# Autodesk Inventor assembly: Assemblyarm
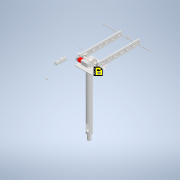
[picture p0: Inventor's stored thumbnail of the model, 180x180]
Saved by Autodesk Inventor 2022 (Build 260153000, 153)
## iProperties
Created: 2022-02-06
Part Number: Assemblyarm
Document SubType Name: Assembly
Designer: pauly
Author: pauly
## Documents named in this file (17)
- C:\Users\pauly\OneDrive\Documents\Robotics arm\Assemblyarm.iam
- C:\Users\pauly\OneDrive\Documents\Robotics arm\Shaft connecting chassis updated 1-19.ipt
- C:\Users\pauly\OneDrive\Documents\Robotics arm\base_plate.ipt
- C:\Users\pauly\OneDrive\Documents\Robotics arm\Updated Support.ipt
- C:\Users\pauly\OneDrive\Documents\Robotics arm\am-2986 FR8ZZ Hex Bearing.ipt
- C:\Users\pauly\OneDrive\Documents\Robotics arm\am-0856 500 Hex Shaft for Modulox REV3.ipt
- C:\Users\pauly\OneDrive\Documents\Robotics arm\arm_plate_btw_support_bicep.ipt
- C:\Users\pauly\OneDrive\Documents\Robotics arm\am-3822 56T 20DP 500hex 375 FW.ipt
- C:\Users\pauly\OneDrive\Documents\Robotics arm\am-3775a_16T 775a RedLine with 16T Pinion.ipt
- C:\Users\pauly\OneDrive\Documents\Robotics arm\am-4212 18T 20DP 500hex 375 FW.ipt
- C:\Users\pauly\OneDrive\Documents\Robotics arm\3 Stage HD - 57 Sport.iam
- C:\Users\pauly\OneDrive\Documents\Robotics arm\am-4457 8 mm ID 22 mm OD Shielded Flanged Bearing F608ZZ.ipt
- C:\Users\pauly\OneDrive\Documents\Robotics arm\1265K67_Rotary Shaft.ipt
- C:\Users\pauly\OneDrive\Documents\Robotics arm\7717N68_MXL Series Lightweight Timing Belt Pulley.ipt
- C:\Users\pauly\OneDrive\Documents\Robotics arm\5202-0002-0051(1)\5202-0002-0051 part.ipt
- C:\Users\pauly\OneDrive\Documents\Robotics arm\7717N25_MXL Series Lightweight Timing Belt Pulley.ipt
- C:\Users\pauly\OneDrive\Documents\Robotics arm\7887K72_MXL Series Timing Belt.ipt
## Components (20 placed, 16 different names)
1. Shaft connecting chassis updated 1-19:1 — Rotational:1
2. base_plate:1 — Rotational:1, Rotational:2, Rotational:3
3. Updated Support:1 — Rotational:2, Rotational:5
4. Updated Support:2 — Rotational:3, Rotational:4
5. am-2986 FR8ZZ Hex Bearing:1 — Rotational:4, Slider:1
6. am-2986 FR8ZZ Hex Bearing:2 — Rotational:5
7. am-0856 500 Hex Shaft for Modulox REV3:1 — Slider:1, Slider:2, Slider:3, Slider:4
8. arm_plate_btw_support_bicep:1 — Slider:2, Rotational:8
9. arm_plate_btw_support_bicep:2 — Slider:3, Rotational:7
10. am-3822 56T 20DP 500hex 375 FW:1 — Slider:4
11. am-3775a_16T 775a RedLine with 16T Pinion:1 — Rotational:6
12. am-4212 18T 20DP 500hex 375 FW:1 — Slider:5
13. 3 Stage HD - 57 Sport:1 [sub-assembly] — Rotational:6, Slider:5
14. am-4457 8 mm ID 22 mm OD Shielded Flanged Bearing F608ZZ:1 — Rotational:7
15. am-4457 8 mm ID 22 mm OD Shielded Flanged Bearing F608ZZ:2 — Rotational:8, Rotational:9
16. 1265K67_Rotary Shaft:1 — Rotational:9, Rotational:10
17. 7717N68_MXL Series Lightweight Timing Belt Pulley:1 — Rotational:10
18. 5202-0002-0051 part:1
19. 7717N25_MXL Series Lightweight Timing Belt Pulley:1
20. 7887K72_MXL Series Timing Belt:1
## Relationships (15: RevoluteJoint 10, TranslationJoint 5)
- Rotational:1 [RevoluteJoint]: Shaft connecting chassis updated 1-19:1 ↔ base_plate:1
- Rotational:2 [RevoluteJoint]: base_plate:1 ↔ Updated Support:1
- Rotational:3 [RevoluteJoint]: base_plate:1 ↔ Updated Support:2
- Rotational:4 [RevoluteJoint]: Updated Support:2 ↔ am-2986 FR8ZZ Hex Bearing:1
- Rotational:5 [RevoluteJoint]: Updated Support:1 ↔ am-2986 FR8ZZ Hex Bearing:2
- Slider:1 [TranslationJoint]: am-2986 FR8ZZ Hex Bearing:1 ↔ am-0856 500 Hex Shaft for Modulox REV3:1
- Slider:2 [TranslationJoint]: am-0856 500 Hex Shaft for Modulox REV3:1 ↔ arm_plate_btw_support_bicep:1
- Slider:3 [TranslationJoint]: am-0856 500 Hex Shaft for Modulox REV3:1 ↔ arm_plate_btw_support_bicep:2
- Slider:4 [TranslationJoint]: am-0856 500 Hex Shaft for Modulox REV3:1 ↔ am-3822 56T 20DP 500hex 375 FW:1
- Rotational:6 [RevoluteJoint]: am-3775a_16T 775a RedLine with 16T Pinion:1 ↔ 3 Stage HD - 57 Sport:1
- Slider:5 [TranslationJoint]: am-4212 18T 20DP 500hex 375 FW:1 ↔ 3 Stage HD - 57 Sport:1
- Rotational:7 [RevoluteJoint]: arm_plate_btw_support_bicep:2 ↔ am-4457 8 mm ID 22 mm OD Shielded Flanged Bearing F608ZZ:1
- Rotational:8 [RevoluteJoint]: arm_plate_btw_support_bicep:1 ↔ am-4457 8 mm ID 22 mm OD Shielded Flanged Bearing F608ZZ:2
- Rotational:9 [RevoluteJoint] (-76.2 mm): am-4457 8 mm ID 22 mm OD Shielded Flanged Bearing F608ZZ:2 ↔ 1265K67_Rotary Shaft:1
- Rotational:10 [RevoluteJoint] (25.4 mm): 1265K67_Rotary Shaft:1 ↔ 7717N68_MXL Series Lightweight Timing Belt Pulley:1
